# Autodesk Inventor assembly: MK-1_Assembly
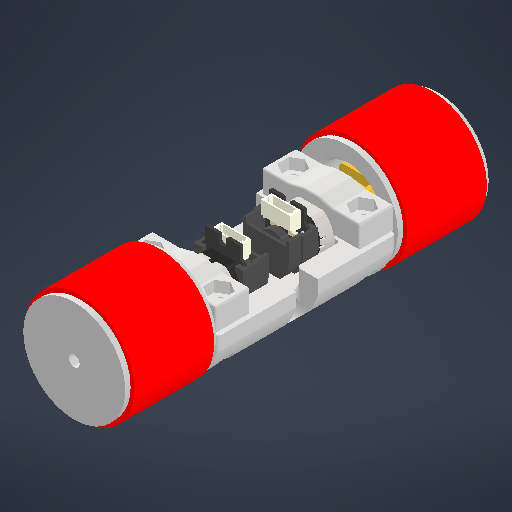
[picture p0: Inventor's stored thumbnail of the model, 512x512]
Saved by Autodesk Inventor 2026.2 (Build 302298010, 298A)
## iProperties
Created: 2026-03-28
Part Number: MK-1_Assembly
Document SubType Name: Assembly
Designer: zak
Author: zak
## Documents named in this file (9)
- C:\Users\zak\GitHub\NeoSumec-MiniSumo-MECH\MK-1_Assembly.iam
- C:\Users\zak\GitHub\NeoSumec-MiniSumo-MECH\_MK-1_\silicon bublebum.ipt
- C:\Users\zak\GitHub\NeoSumec-MiniSumo-MECH\_MK-1_\Wheel.ipt
- C:\Users\zak\GitHub\NeoSumec-MiniSumo-MECH\_MK-1_\Pololu Micro Metal Gearmotor 3D (STEP) Models\With Encoder, Side Connector\mmgm-cb-enc-side-con\mmgm-cb-enc-side-con\mmgm-cb-enc-side-con.ipt
- C:\Users\zak\GitHub\NeoSumec-MiniSumo-MECH\_MK-1_\silicon bublebum_MIR.ipt
- C:\Users\zak\GitHub\NeoSumec-MiniSumo-MECH\_MK-1_\Wheel_MIR.ipt
- C:\Users\zak\GitHub\NeoSumec-MiniSumo-MECH\_MK-1_\Pololu Micro Metal Gearmotor 3D (STEP) Models\With Encoder, Side Connector\mmgm-cb-enc-side-con\mmgm-cb-enc-side-con\mmgm-cb-enc-side-con_MIR.ipt
- C:\Users\zak\GitHub\NeoSumec-MiniSumo-MECH\_MK-1_\MotorMountBottom.ipt
- C:\Users\zak\GitHub\NeoSumec-MiniSumo-MECH\_MK-1_\MotorClamp.ipt
## Components (9 placed, 8 different names)
1. silicon bublebum:1 — Proti sobě:1, Proti sobě:2
2. Wheel:1 — Proti sobě:1, Proti sobě:2, Proti sobě:3, Proti sobě:4, Proti sobě:11
3. mmgm-cb-enc-side-con:1 — Proti sobě:3, Proti sobě:4, Stejný směr:1, Proti sobě:9, Proti sobě:10
4. silicon bublebum_MIR:1 — Proti sobě:5, Proti sobě:6
5. Wheel_MIR:1 — Proti sobě:5, Proti sobě:6, Proti sobě:7, Proti sobě:8, Proti sobě:12
6. mmgm-cb-enc-side-con_MIR:1 — Proti sobě:7, Proti sobě:8, Stejný směr:1, Proti sobě:9, Stejný směr:2
7. MotorMountBottom:1 — Proti sobě:10, Stejný směr:2, Proti sobě:11, Proti sobě:12, Proti sobě:13, Proti sobě:14, Proti sobě:15, Proti sobě:16, Proti sobě:17, Proti sobě:18
8. MotorClamp:1 — Proti sobě:13, Proti sobě:14, Proti sobě:15
9. MotorClamp:2 — Proti sobě:16, Proti sobě:17, Proti sobě:18
## Relationships (20: Mate 18, Flush 2)
- Proti sobě:1 [Mate]: silicon bublebum:1 ↔ Wheel:1
- Proti sobě:2 [Mate]: silicon bublebum:1 ↔ Wheel:1
- Proti sobě:3 [Mate]: Wheel:1 ↔ mmgm-cb-enc-side-con:1
- Proti sobě:4 [Mate] (0.25 mm): Wheel:1 ↔ mmgm-cb-enc-side-con:1
- Proti sobě:5 [Mate]: silicon bublebum_MIR:1 ↔ Wheel_MIR:1
- Proti sobě:6 [Mate]: silicon bublebum_MIR:1 ↔ Wheel_MIR:1
- Proti sobě:7 [Mate] (0.25 mm): Wheel_MIR:1 ↔ mmgm-cb-enc-side-con_MIR:1
- Proti sobě:8 [Mate]: Wheel_MIR:1 ↔ mmgm-cb-enc-side-con_MIR:1
- Stejný směr:1 [Flush]: mmgm-cb-enc-side-con:1 ↔ mmgm-cb-enc-side-con_MIR:1
- Proti sobě:9 [Mate]: mmgm-cb-enc-side-con:1 ↔ mmgm-cb-enc-side-con_MIR:1
- Proti sobě:10 [Mate]: mmgm-cb-enc-side-con:1 ↔ MotorMountBottom:1
- Stejný směr:2 [Flush] (8 mm): mmgm-cb-enc-side-con_MIR:1 ↔ MotorMountBottom:1
- Proti sobě:11 [Mate] (0.5 mm): Wheel:1 ↔ MotorMountBottom:1
- Proti sobě:12 [Mate] (0.5 mm): Wheel_MIR:1 ↔ MotorMountBottom:1
- Proti sobě:13 [Mate]: MotorMountBottom:1 ↔ MotorClamp:1
- Proti sobě:14 [Mate]: MotorMountBottom:1 ↔ MotorClamp:1
- Proti sobě:15 [Mate] (0.75 mm): MotorMountBottom:1 ↔ MotorClamp:1
- Proti sobě:16 [Mate]: MotorMountBottom:1 ↔ MotorClamp:2
- Proti sobě:17 [Mate]: MotorMountBottom:1 ↔ MotorClamp:2
- Proti sobě:18 [Mate] (0.75 mm): MotorMountBottom:1 ↔ MotorClamp:2
